# Autodesk Inventor assembly: Jadi1
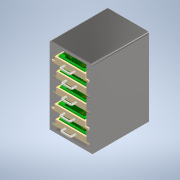
[picture p0: Inventor's stored thumbnail of the model, 180x180]
Saved by Autodesk Inventor 2021 (Build 250183000, 183)
## iProperties
Created: 2023-04-06
Part Number: Jadi1
Document SubType Name: Assembly
Designer: EF0481
Author: EF0481
## Documents named in this file (6)
- C:\Users\EF0481\Documents\3D\Jadi1.iam
- C:\Users\EF0481\Documents\3D\Slider_tatak.ipt
- C:\Users\EF0481\Documents\3D\Gagang.ipt
- C:\Users\EF0481\Documents\3D\PCB.ipt
- C:\Users\EF0481\Documents\3D\RackV2.ipt
- C:\Users\EF0481\Documents\3D\backdor.ipt
## Components (17 placed, 5 different names)
1. RackV2:1 — Mate:10, Mate:11, Mate:21, Mate:22, Mate:23, Mate:24, Mate:25, Mate:26, Mate:27, Mate:28, Mate:29, Mate:30, Mate:31, Mate:32, Mate:33
2. Slider_tatak:2 — Mate:10, Mate:11
3. Gagang:2
4. PCB:2
5. Slider_tatak:3 — Mate:21, Mate:22
6. Gagang:3
7. PCB:3
8. Slider_tatak:4 — Mate:25, Mate:26
9. Gagang:4
10. PCB:4
11. Slider_tatak:5 — Mate:27, Mate:28
12. Gagang:5
13. PCB:5
14. Slider_tatak:6 — Mate:23, Mate:24
15. Gagang:6
16. PCB:6
17. backdor:1 — Mate:29, Mate:30, Mate:31, Mate:32, Mate:33
## Relationships (35: Mate 30, WeldJoint 5)
- [WeldJoint]: Slider_tatak:2 ↔ PCB:2
- [Mate]: Slider_tatak:2 ↔ Gagang:2
- [Mate]: Slider_tatak:2 ↔ Gagang:2
- [Mate]: Slider_tatak:2 ↔ Gagang:2
- [WeldJoint]: Slider_tatak:3 ↔ PCB:3
- [Mate]: Slider_tatak:3 ↔ Gagang:3
- [Mate]: Slider_tatak:3 ↔ Gagang:3
- [Mate]: Slider_tatak:3 ↔ Gagang:3
- Mate:10: RackV2:1 ↔ Slider_tatak:2
- Mate:11: RackV2:1 ↔ Slider_tatak:2
- [WeldJoint]: Slider_tatak:4 ↔ PCB:4
- [Mate]: Slider_tatak:4 ↔ Gagang:4
- [Mate]: Slider_tatak:4 ↔ Gagang:4
- [Mate]: Slider_tatak:4 ↔ Gagang:4
- [WeldJoint]: Slider_tatak:5 ↔ PCB:5
- [Mate]: Slider_tatak:5 ↔ Gagang:5
- [Mate]: Slider_tatak:5 ↔ Gagang:5
- [Mate]: Slider_tatak:5 ↔ Gagang:5
- [WeldJoint]: Slider_tatak:6 ↔ PCB:6
- [Mate]: Slider_tatak:6 ↔ Gagang:6
- [Mate]: Slider_tatak:6 ↔ Gagang:6
- [Mate]: Slider_tatak:6 ↔ Gagang:6
- Mate:21: RackV2:1 ↔ Slider_tatak:3
- Mate:22: RackV2:1 ↔ Slider_tatak:3
- Mate:23: RackV2:1 ↔ Slider_tatak:6
- Mate:24: RackV2:1 ↔ Slider_tatak:6
- Mate:25: RackV2:1 ↔ Slider_tatak:4
- Mate:26: RackV2:1 ↔ Slider_tatak:4
- Mate:27: RackV2:1 ↔ Slider_tatak:5
- Mate:28: RackV2:1 ↔ Slider_tatak:5
- Mate:29: RackV2:1 ↔ backdor:1
- Mate:30: RackV2:1 ↔ backdor:1
- Mate:31: RackV2:1 ↔ backdor:1
- Mate:32: RackV2:1 ↔ backdor:1
- Mate:33: RackV2:1 ↔ backdor:1
## Named parameters: d78_d77 = 0 mm, d79_d74 = 0 mm, d80_d75 = 0 mm, d81_d76 = 0 mm, d84_d78_d77 = 0 mm, d85_d79_d74 = 0 mm, d86_d80_d75 = 0 mm, d87_d81_d76 = 0 mm, d90_d84_d78_d77 = 0 mm, d91_d85_d79_d74 = 0 mm, d92_d86_d80_d75 = 0 mm, d93_d87_d81_d76 = 0 mm, d94_d90_d84_d78_d77 = 0 mm, d95_d91_d85_d79_d74 = 0 mm, d96_d92_d86_d80_d75 = 0 mm, d97_d93_d87_d81_d76 = 0 mm, d98_d90_d84_d78_d77 = 0 mm, d99_d91_d85_d79_d74 = 0 mm, d100_d92_d86_d80_d75 = 0 mm, d101_d93_d87_d81_d76 = 0 mm
